# Autodesk Inventor assembly: gear_clutch
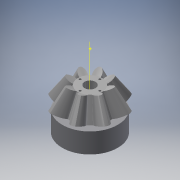
[picture p0: Inventor's stored thumbnail of the model, 180x180]
Saved by Autodesk Inventor 2018 (Build 220112000, 112)
## iProperties
Created: 2018-08-10
Part Number: gear_clutch
Document SubType Name: Assembly
Designer: Bardo91
Author: Bardo91
## Documents named in this file (3)
- D:\programming\hecatonquiros\cad_models\accesories\gripper_clutch\gear_clutch.iam
- D:\programming\hecatonquiros\cad_models\accesories\gripper_clutch\Bevel Gear12.ipt
- D:\programming\hecatonquiros\cad_models\accesories\gripper_clutch\embrague_1.ipt
## Components (2 placed, 2 different names)
1. Bevel Gear1:1 — Mate:1, Mate:2
2. embrague_1:1 — Mate:1, Mate:2
## Relationships (2: Mate 2)
- Mate:1: Bevel Gear1:1 ↔ embrague_1:1
- Mate:2: Bevel Gear1:1 ↔ embrague_1:1
